# Autodesk Inventor assembly: MIR6x1inTractionWheel-1111-2016
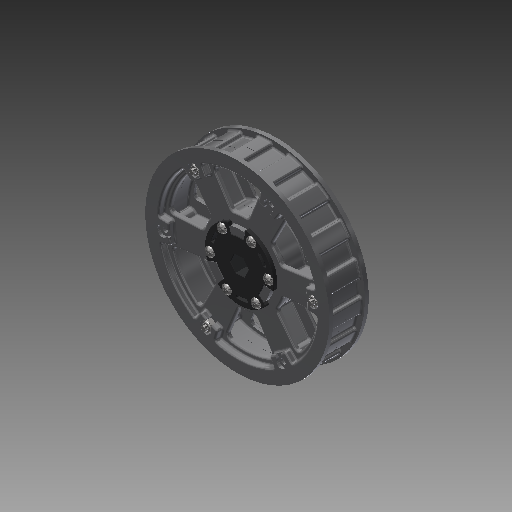
[picture p0: Inventor's stored thumbnail of the model, 512x512]
Saved by Autodesk Inventor 2017 (Build 210142000, 142)
## iProperties
Created: 2016-12-09
Part Number: MIR6x1inTractionWheel-1111-2016
Document SubType Name: Assembly
Designer: Phyllis
Author: smiku
## Documents named in this file (8)
- E:\GrabCAD\Power Hawks CAD\Resources\VEXpro Resources\Wheels\6 inch\MIR6x1inTractionWheel-1111-2016.iam
- E:\GrabCAD\Power Hawks CAD\Resources\VEXpro Resources\Wheels\Wheel Parts\MIR6InchWheelEnd-1111-20161.ipt
- E:\GrabCAD\Power Hawks CAD\Resources\VEXpro Resources\Fasteners\Standoffs\MIRStandoff0.75in-1111-20161.ipt
- E:\GrabCAD\Power Hawks CAD\Resources\VEXpro Resources\Versa Motion\MIRVersaHub(0.5inHex)-1111-20161.ipt
- E:\GrabCAD\Power Hawks CAD\Resources\VEXpro Resources\Versa Motion\MIRVersaHub(0.5inHex,Plastic)-1111-20161.ipt
- E:\GrabCAD\Power Hawks CAD\Resources\VEXpro Resources\Fasteners\Screws\MIRScrew8-32x1.25in-1111-20161.ipt
- E:\GrabCAD\Power Hawks CAD\Resources\VEXpro Resources\Fasteners\Screws\MIRScrew8-32x0.5in-1111-20161.ipt
- E:\GrabCAD\Power Hawks CAD\Resources\VEXpro Resources\Fasteners\Nuts\MIRNut8-32Nylock-1111-20161.ipt
## Components (28 placed, 7 different names)
1. MIR6InchWheelEnd-1111-20161:1 — Angle:1, Angle:3, Insert:17, Angle:4, Insert:16, Angle:2, Insert:18, Rotational:1, Rotational:9, Rotational:8, Rotational:7, Rotational:6
2. MIR6InchWheelEnd-1111-20161:2 — Insert:1, Insert:2, Insert:3, Rotational:9, Rotational:8, Rotational:5, Rotational:4
3. MIRVersaHub(0.5inHex)-1111-20161:1 — Insert:9, Insert:8, Insert:7, Insert:6, Insert:5, Insert:4, Rotational:5, Rotational:4
4. MIRVersaHub(0.5inHex,Plastic)-1111-20161:1 — Insert:10, Insert:11, Insert:12, Insert:13, Insert:14, Insert:15, Rotational:7, Rotational:6
5. MIRScrew8-32x1.25in-1111-20161:1 — Insert:1
6. MIRScrew8-32x1.25in-1111-20161:2 — Insert:2
7. MIRScrew8-32x1.25in-1111-20161:3 — Insert:3
8. MIRScrew8-32x0.5in-1111-20161:1 — Insert:9
9. MIRScrew8-32x0.5in-1111-20161:2 — Insert:8
10. MIRScrew8-32x0.5in-1111-20161:3 — Insert:7
11. MIRScrew8-32x0.5in-1111-20161:4 — Insert:6
12. MIRScrew8-32x0.5in-1111-20161:5 — Insert:5
13. MIRScrew8-32x0.5in-1111-20161:6 — Insert:4
14. MIRScrew8-32x0.5in-1111-20161:7 — Insert:10
15. MIRScrew8-32x0.5in-1111-20161:8 — Insert:11
16. MIRScrew8-32x0.5in-1111-20161:9 — Insert:12
17. MIRScrew8-32x0.5in-1111-20161:10 — Insert:13
18. MIRScrew8-32x0.5in-1111-20161:11 — Insert:14
19. MIRScrew8-32x0.5in-1111-20161:12 — Insert:15
20. MIRNut8-32Nylock-1111-20161:1 — Angle:3, Insert:17
21. MIRNut8-32Nylock-1111-20161:2 — Angle:4, Insert:16
22. MIRNut8-32Nylock-1111-20161:3 — Angle:2, Insert:18
23. MIRStandoff0.75in-1111-20161:1 — Angle:1, Rotational:1
24. MIRStandoff0.75in-1111-20161:2
25. MIRStandoff0.75in-1111-20161:3
26. MIRStandoff0.75in-1111-20161:4
27. MIRStandoff0.75in-1111-20161:5
28. MIRStandoff0.75in-1111-20161:6
## Component patterns: (6 elements, first: MIRStandoff0.75in-1111-20161:1)
## Relationships (29: Insert 18, RevoluteJoint 7, Angle 4)
- Angle:1 (0 deg): MIR6InchWheelEnd-1111-20161:1 ↔ MIRStandoff0.75in-1111-20161:1
- Insert:1: MIR6InchWheelEnd-1111-20161:2 ↔ MIRScrew8-32x1.25in-1111-20161:1
- Insert:2: MIR6InchWheelEnd-1111-20161:2 ↔ MIRScrew8-32x1.25in-1111-20161:2
- Insert:3: MIR6InchWheelEnd-1111-20161:2 ↔ MIRScrew8-32x1.25in-1111-20161:3
- Insert:9: MIRVersaHub(0.5inHex)-1111-20161:1 ↔ MIRScrew8-32x0.5in-1111-20161:1
- Insert:8: MIRVersaHub(0.5inHex)-1111-20161:1 ↔ MIRScrew8-32x0.5in-1111-20161:2
- Insert:7: MIRVersaHub(0.5inHex)-1111-20161:1 ↔ MIRScrew8-32x0.5in-1111-20161:3
- Insert:6: MIRVersaHub(0.5inHex)-1111-20161:1 ↔ MIRScrew8-32x0.5in-1111-20161:4
- Insert:5: MIRVersaHub(0.5inHex)-1111-20161:1 ↔ MIRScrew8-32x0.5in-1111-20161:5
- Insert:4: MIRVersaHub(0.5inHex)-1111-20161:1 ↔ MIRScrew8-32x0.5in-1111-20161:6
- Insert:10: MIRVersaHub(0.5inHex,Plastic)-1111-20161:1 ↔ MIRScrew8-32x0.5in-1111-20161:7
- Insert:11: MIRVersaHub(0.5inHex,Plastic)-1111-20161:1 ↔ MIRScrew8-32x0.5in-1111-20161:8
- Insert:12: MIRVersaHub(0.5inHex,Plastic)-1111-20161:1 ↔ MIRScrew8-32x0.5in-1111-20161:9
- Insert:13: MIRVersaHub(0.5inHex,Plastic)-1111-20161:1 ↔ MIRScrew8-32x0.5in-1111-20161:10
- Insert:14: MIRVersaHub(0.5inHex,Plastic)-1111-20161:1 ↔ MIRScrew8-32x0.5in-1111-20161:11
- Insert:15: MIRVersaHub(0.5inHex,Plastic)-1111-20161:1 ↔ MIRScrew8-32x0.5in-1111-20161:12
- Angle:3 (0 deg): MIR6InchWheelEnd-1111-20161:1 ↔ MIRNut8-32Nylock-1111-20161:1
- Insert:17: MIR6InchWheelEnd-1111-20161:1 ↔ MIRNut8-32Nylock-1111-20161:1
- Angle:4 (0 deg): MIR6InchWheelEnd-1111-20161:1 ↔ MIRNut8-32Nylock-1111-20161:2
- Insert:16: MIR6InchWheelEnd-1111-20161:1 ↔ MIRNut8-32Nylock-1111-20161:2
- Angle:2 (0 deg): MIR6InchWheelEnd-1111-20161:1 ↔ MIRNut8-32Nylock-1111-20161:3
- Insert:18: MIR6InchWheelEnd-1111-20161:1 ↔ MIRNut8-32Nylock-1111-20161:3
- Rotational:1 [RevoluteJoint]: MIR6InchWheelEnd-1111-20161:1 ↔ MIRStandoff0.75in-1111-20161:1
- Rotational:9 [RevoluteJoint]: MIR6InchWheelEnd-1111-20161:1 ↔ MIR6InchWheelEnd-1111-20161:2
- Rotational:8 [RevoluteJoint]: MIR6InchWheelEnd-1111-20161:1 ↔ MIR6InchWheelEnd-1111-20161:2
- Rotational:5 [RevoluteJoint]: MIR6InchWheelEnd-1111-20161:2 ↔ MIRVersaHub(0.5inHex)-1111-20161:1
- Rotational:4 [RevoluteJoint]: MIR6InchWheelEnd-1111-20161:2 ↔ MIRVersaHub(0.5inHex)-1111-20161:1
- Rotational:7 [RevoluteJoint]: MIR6InchWheelEnd-1111-20161:1 ↔ MIRVersaHub(0.5inHex,Plastic)-1111-20161:1
- Rotational:6 [RevoluteJoint]: MIR6InchWheelEnd-1111-20161:1 ↔ MIRVersaHub(0.5inHex,Plastic)-1111-20161:1
